# Autodesk Inventor assembly: HexaBot
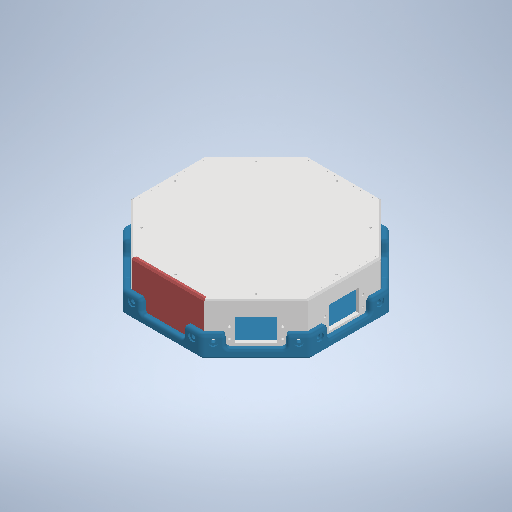
[picture p0: Inventor's stored thumbnail of the model, 512x512]
Saved by Autodesk Inventor 2025.1 (Build 291241020, 241B)
## iProperties
Created: 2024-08-28
Part Number: HexaBot
Document SubType Name: Assembly
Designer: SEON06
Author: SEON06
## Documents named in this file (5)
- C:\Users\daare\Documents\Inventor\HexaBot_s\HexaBot.iam
- C:\Users\daare\Documents\Inventor\HexaBot_s\Base.ipt
- C:\Users\daare\Documents\Inventor\HexaBot_s\Wall.ipt
- C:\Users\daare\Documents\Inventor\HexaBot_s\Cap.ipt
- C:\Users\daare\Documents\Inventor\HexaBot_s\Wall-for-Motor.ipt
## Components (10 placed, 4 different names)
1. Base:1 — 메이트:1, 각도:1, 메이트:2, 메이트:3, 메이트:7, 메이트:13, 메이트:18, 메이트:23, 메이트:24, 메이트:25, 메이트:26, 메이트:27, 메이트:28, 메이트:29, 메이트:30, 메이트:31, 메이트:32, 메이트:33, 메이트:34, 메이트:35, 메이트:36, 메이트:37, 메이트:38, 메이트:39, 메이트:40
2. Wall:1 — 메이트:2, 메이트:3, 메이트:7, 대칭:2, 메이트:22
3. Wall:5 — 메이트:13, 메이트:18, 대칭:2
4. Cap:1 — 메이트:22
5. Wall-for-Motor:1 — 메이트:23, 메이트:24, 메이트:25
6. Wall-for-Motor:2 — 메이트:26, 메이트:27, 메이트:28
7. Wall-for-Motor:3 — 메이트:29, 메이트:30, 메이트:31
8. Wall-for-Motor:4 — 메이트:35, 메이트:36, 메이트:37
9. Wall-for-Motor:5 — 메이트:32, 메이트:33, 메이트:34
10. Wall-for-Motor:6 — 메이트:38, 메이트:39, 메이트:40
## Relationships (27: Mate 25, Angle 1, Symmetry 1)
- 메이트:1 [Mate]: Base:1
- 각도:1 [Angle] (0 deg): Base:1
- 메이트:2 [Mate]: Base:1 ↔ Wall:1
- 메이트:3 [Mate]: Base:1 ↔ Wall:1
- 메이트:7 [Mate]: Base:1 ↔ Wall:1
- 메이트:13 [Mate]: Base:1 ↔ Wall:5
- 메이트:18 [Mate]: Base:1 ↔ Wall:5
- 대칭:2 [Symmetry]: Wall:1 ↔ Wall:5
- 메이트:22 [Mate]: Wall:1 ↔ Cap:1
- 메이트:23 [Mate]: Base:1 ↔ Wall-for-Motor:1
- 메이트:24 [Mate]: Base:1 ↔ Wall-for-Motor:1
- 메이트:25 [Mate]: Base:1 ↔ Wall-for-Motor:1
- 메이트:26 [Mate]: Base:1 ↔ Wall-for-Motor:2
- 메이트:27 [Mate]: Base:1 ↔ Wall-for-Motor:2
- 메이트:28 [Mate]: Base:1 ↔ Wall-for-Motor:2
- 메이트:29 [Mate]: Base:1 ↔ Wall-for-Motor:3
- 메이트:30 [Mate]: Base:1 ↔ Wall-for-Motor:3
- 메이트:31 [Mate]: Base:1 ↔ Wall-for-Motor:3
- 메이트:32 [Mate]: Base:1 ↔ Wall-for-Motor:5
- 메이트:33 [Mate]: Base:1 ↔ Wall-for-Motor:5
- 메이트:34 [Mate]: Base:1 ↔ Wall-for-Motor:5
- 메이트:35 [Mate]: Base:1 ↔ Wall-for-Motor:4
- 메이트:36 [Mate]: Base:1 ↔ Wall-for-Motor:4
- 메이트:37 [Mate]: Base:1 ↔ Wall-for-Motor:4
- 메이트:38 [Mate]: Base:1 ↔ Wall-for-Motor:6
- 메이트:39 [Mate]: Base:1 ↔ Wall-for-Motor:6
- 메이트:40 [Mate]: Base:1 ↔ Wall-for-Motor:6
